# Autodesk Inventor assembly: BtnHolder
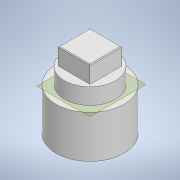
[picture p0: Inventor's stored thumbnail of the model, 180x180]
Saved by Autodesk Inventor 2021 (Build 250183000, 183)
## iProperties
Created: 2021-08-30
Part Number: BtnHolder
Document SubType Name: Assembly
Designer: teh18
Author: teh18
## Documents named in this file (3)
- C:\Users\teh18\OneDrive\BVE Controller\r68-bve-mascon\handle-base\BtnHolder.iam
- C:\Users\teh18\OneDrive\BVE Controller\r68-bve-mascon\D6C90 F1 LFS.ipt
- C:\Users\teh18\OneDrive\BVE Controller\r68-bve-mascon\handle-base\BtnHolder.ipt
## Components (2 placed, 2 different names)
1. D6C90 F1 LFS:1 — Flush:1, Mate:1
2. BtnHolder:1 — Flush:1, Mate:1
## Relationships (2: Flush 1, Mate 1)
- Flush:1: D6C90 F1 LFS:1 ↔ BtnHolder:1
- Mate:1: D6C90 F1 LFS:1 ↔ BtnHolder:1
